# Autodesk Inventor assembly: rigt_motor_asembly
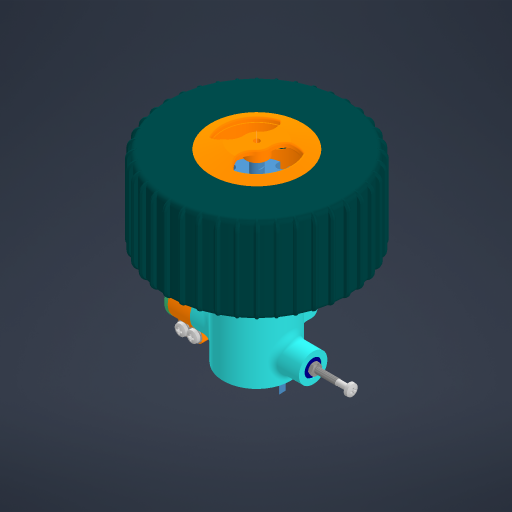
[picture p0: Inventor's stored thumbnail of the model, 512x512]
Saved by Autodesk Inventor 2024 (Build 280153000, 153)
## iProperties
Created: 2023-05-14
Part Number: rigt_motor_asembly
Document SubType Name: Assembly
Designer: user
Mass: 529.807 g
Surface Area: 912.469 cm^2
Volume: 506.199 cm^3
Density: 1.04664 g/cm^3
Author: user
## Documents named in this file (14)
- D:\Docs\Robot\3d\motor_assembly\left_motor_asembly.iam
- D:\Docs\Robot\3d\motor_assembly\bushing_assembly.iam
- D:\Docs\Robot\3d\default_components\motor.ipt
- D:\Docs\Robot\3d\default_components\wheel.ipt
- D:\Docs\Robot\3d\default_components\604zz_bearing.ipt
- C:\Users\user\Documents\Inventor\Content Center Files\R2024\ru-RU\DIN 934\DIN 934 - M4 x 0,7.ipt
- D:\Docs\Robot\3d\motor_assembly\default_motor_asembly\cup.ipt
- D:\Docs\Robot\3d\motor_assembly\left_motor_asembly\lower_arm.ipt
- C:\Users\user\Documents\Inventor\Content Center Files\R2024\ru-RU\DIN 7985 (H)\DIN 7985 (H) - M4x30-H.ipt
- C:\Users\user\Documents\Inventor\Content Center Files\R2024\ru-RU\DIN 125-1  A\DIN 125 - A 4,3.ipt
- C:\Users\user\Documents\Inventor\Content Center Files\R2024\ru-RU\DIN 7985 (H)\DIN 7985 (H) - M4x20-H.ipt
- C:\Users\user\Documents\Inventor\Content Center Files\R2024\ru-RU\DIN 7985 (H)\DIN 7985 (H) - M3x20-H.ipt
- C:\Users\user\Documents\Inventor\Content Center Files\R2024\ru-RU\DIN 934\DIN 934 - M3 x 0,5.ipt
- D:\Docs\Robot\3d_v2\machine_body\wheel_assembly.iam
## Components (27 placed, 13 different names)
1. lower_arm:2 — Вставка:11, Вставка:15, Вставка:17, Вставка:18, Вставка:19, Вставка:20, Вставка:21, Вставка:22, Вставка:35, Вставка:36, Вставка:37
2. bushing_assembly:2 [sub-assembly] — Вставка:37
3. motor:1 — Вставка:4, Вставка:11, Вставка:38
4. wheel:1 — Вставка:4
5. 604zz_bearing:1 — Вставка:8, Вставка:15, Вставка:16
6. DIN 934 - заменено на DIN EN 24032/28673/28674 M4:1 — Вставка:8
7. cup:1 — Вставка:17, Вставка:18, Вставка:23, Вставка:24, Вставка:25, Вставка:26
8. DIN 7985 (H) M4x30-H:1 — Вставка:16
9. DIN 125-1 A A 4,3:1 — Вставка:19, Вставка:33
10. DIN 125-1 A A 4,3:2 — Вставка:20, Вставка:32
11. DIN 125-1 A A 4,3:3 — Вставка:21, Вставка:31
12. DIN 125-1 A A 4,3:4 — Вставка:24, Вставка:27
13. DIN 125-1 A A 4,3:5 — Вставка:22, Вставка:34
14. DIN 125-1 A A 4,3:6 — Вставка:25, Вставка:29
15. DIN 125-1 A A 4,3:7 — Вставка:26, Вставка:30
16. DIN 125-1 A A 4,3:8 — Вставка:23, Вставка:28
17. DIN 7985 (H) M4x20-H:1 — Вставка:27
18. DIN 7985 (H) M4x20-H:2 — Вставка:30
19. DIN 7985 (H) M4x20-H:3 — Вставка:28
20. DIN 7985 (H) M4x20-H:4 — Вставка:29
21. DIN 934 - заменено на DIN EN 24032/28673/28674 M4:2 — Вставка:31
22. DIN 934 - заменено на DIN EN 24032/28673/28674 M4:3 — Вставка:32
23. DIN 934 - заменено на DIN EN 24032/28673/28674 M4:4 — Вставка:33
24. DIN 934 - заменено на DIN EN 24032/28673/28674 M4:5 — Вставка:34
25. DIN 7985 (H) M3x20-H:1 — Вставка:35
26. DIN 934 - заменено на DIN EN 24032/28673/28674 M3:1 — Вставка:36
27. wheel_assembly:1 [sub-assembly] — Вставка:38
## Relationships (31: Insert 27, Mate 4)
- [Mate]: lower_arm:2
- [Mate]: lower_arm:2
- [Mate]: lower_arm:2
- Вставка:4 [Insert]: motor:1 ↔ wheel:1
- [Mate]: lower_arm:2
- Вставка:8 [Insert]: 604zz_bearing:1 ↔ DIN 934 - заменено на DIN EN 24032/28673/28674 M4:1
- Вставка:11 [Insert]: lower_arm:2 ↔ motor:1
- Вставка:15 [Insert]: lower_arm:2 ↔ 604zz_bearing:1
- Вставка:16 [Insert]: 604zz_bearing:1 ↔ DIN 7985 (H) M4x30-H:1
- Вставка:17 [Insert]: lower_arm:2 ↔ cup:1
- Вставка:18 [Insert]: lower_arm:2 ↔ cup:1
- Вставка:19 [Insert]: lower_arm:2 ↔ DIN 125-1 A A 4,3:1
- Вставка:20 [Insert]: lower_arm:2 ↔ DIN 125-1 A A 4,3:2
- Вставка:21 [Insert]: lower_arm:2 ↔ DIN 125-1 A A 4,3:3
- Вставка:22 [Insert]: lower_arm:2 ↔ DIN 125-1 A A 4,3:5
- Вставка:23 [Insert]: cup:1 ↔ DIN 125-1 A A 4,3:8
- Вставка:24 [Insert]: cup:1 ↔ DIN 125-1 A A 4,3:4
- Вставка:25 [Insert]: cup:1 ↔ DIN 125-1 A A 4,3:6
- Вставка:26 [Insert]: cup:1 ↔ DIN 125-1 A A 4,3:7
- Вставка:27 [Insert]: DIN 125-1 A A 4,3:4 ↔ DIN 7985 (H) M4x20-H:1
- Вставка:28 [Insert]: DIN 125-1 A A 4,3:8 ↔ DIN 7985 (H) M4x20-H:3
- Вставка:29 [Insert]: DIN 125-1 A A 4,3:6 ↔ DIN 7985 (H) M4x20-H:4
- Вставка:30 [Insert]: DIN 125-1 A A 4,3:7 ↔ DIN 7985 (H) M4x20-H:2
- Вставка:31 [Insert]: DIN 125-1 A A 4,3:3 ↔ DIN 934 - заменено на DIN EN 24032/28673/28674 M4:2
- Вставка:32 [Insert]: DIN 125-1 A A 4,3:2 ↔ DIN 934 - заменено на DIN EN 24032/28673/28674 M4:3
- Вставка:33 [Insert]: DIN 125-1 A A 4,3:1 ↔ DIN 934 - заменено на DIN EN 24032/28673/28674 M4:4
- Вставка:34 [Insert]: DIN 125-1 A A 4,3:5 ↔ DIN 934 - заменено на DIN EN 24032/28673/28674 M4:5
- Вставка:35 [Insert]: lower_arm:2 ↔ DIN 7985 (H) M3x20-H:1
- Вставка:36 [Insert]: lower_arm:2 ↔ DIN 934 - заменено на DIN EN 24032/28673/28674 M3:1
- Вставка:37 [Insert]: lower_arm:2 ↔ bushing_assembly:2
- Вставка:38 [Insert]: motor:1 ↔ wheel_assembly:1
